# Autodesk Inventor assembly: GANTRY
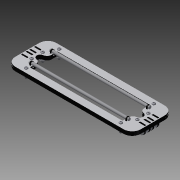
[picture p0: Inventor's stored thumbnail of the model, 180x180]
Saved by Autodesk Inventor 2013 (Build 170138000, 138)
## iProperties
Created: 2014-06-21
Part Number: GANTRY
Document SubType Name: Assembly
Designer: employee
Author: employee
## Documents named in this file (11)
- C:\Users\employee\Desktop\CoreXZ 2\GANTRY.iam
- C:\Users\employee\Desktop\CoreXZ 2\GANTRY BACK.ipt
- C:\Users\employee\Desktop\CoreXZ 2\GANTRY FRONT.ipt
- C:\Users\employee\Desktop\CoreXZ 2\M8X290 ROD.ipt
- C:\Users\employee\Desktop\CoreXZ 2\LM8UU.ipt
- C:\Users\employee\Desktop\CoreXZ 2\625vv.ipt
- C:\Users\employee\Desktop\CoreXZ 2\M5 WASHER.ipt
- C:\Users\employee\Desktop\CoreXZ 2\M5 NUT.ipt
- C:\Users\employee\Desktop\CoreXZ 2\M5X25.ipt
- C:\Users\employee\Desktop\CoreXZ 2\ZIP TIE GANTRY ROD.ipt
- C:\Users\employee\Desktop\CoreXZ 2\ZIP TIE GANTRY BEARING.ipt
## Components (52 placed, 10 different names)
1. GANTRY BACK:1 — Insert:1, Insert:2, Mate:4, Mate:5, Tangent:5, Tangent:6, Tangent:7, Tangent:8, Angle:5, Angle:6, Angle:7, Angle:8, Angle:9, Angle:10, Angle:11, Angle:12, Insert:65, Insert:66, Insert:67, Insert:68, Insert:69, Insert:70, Insert:71, Insert:72
2. GANTRY FRONT:1 — Insert:1, Insert:2, Mate:2, Tangent:1, Tangent:2, Mate:3, Tangent:3, Tangent:4, Angle:1, Angle:2, Angle:3, Angle:4, Insert:73, Insert:74, Insert:75, Insert:76, Insert:77, Insert:78, Insert:79, Insert:80
3. M8X290 ROD:2 — Mate:2, Tangent:1, Tangent:2, Insert:38, Insert:40
4. M8X290 ROD:3 — Mate:3, Tangent:3, Tangent:4, Insert:37, Insert:39
5. LM8UU:1 — Insert:35, Mate:4, Tangent:7, Tangent:8, Insert:47, Insert:48
6. LM8UU:2 — Insert:35, Insert:45, Insert:46
7. LM8UU:3 — Insert:36, Mate:5, Tangent:5, Tangent:6, Insert:43, Insert:44
8. LM8UU:4 — Insert:36, Insert:41, Insert:42
9. ZIP TIE GANTRY ROD:1 — Insert:37, Angle:3
10. ZIP TIE GANTRY ROD:2 — Insert:40, Angle:2
11. ZIP TIE GANTRY ROD:3 — Insert:39, Angle:1
12. ZIP TIE GANTRY ROD:4 — Insert:38, Angle:4
13. ZIP TIE GANTRY BEARING:1 — Insert:41, Angle:5
14. ZIP TIE GANTRY BEARING:2 — Insert:42, Angle:6
15. ZIP TIE GANTRY BEARING:3 — Insert:43, Angle:8
16. ZIP TIE GANTRY BEARING:4 — Insert:44, Angle:7
17. ZIP TIE GANTRY BEARING:5 — Insert:45, Angle:12
18. ZIP TIE GANTRY BEARING:6 — Insert:46, Angle:11
19. ZIP TIE GANTRY BEARING:7 — Insert:47, Angle:9
20. ZIP TIE GANTRY BEARING:8 — Insert:48, Angle:10
21. 625vv:1 — Insert:49, Insert:57
22. M5 NUT:1 — Insert:57
23. M5 WASHER:1 — Insert:49, Insert:65
24. 625vv:2 — Insert:50, Insert:58
25. M5 NUT:2 — Insert:58
26. M5 WASHER:2 — Insert:50, Insert:66
27. 625vv:3 — Insert:51, Insert:59
28. M5 NUT:3 — Insert:59
29. M5 WASHER:3 — Insert:51, Insert:67
30. 625vv:4 — Insert:52, Insert:60
31. M5 NUT:4 — Insert:60
32. M5 WASHER:4 — Insert:52, Insert:68
33. 625vv:5 — Insert:53, Insert:61
34. M5 NUT:5 — Insert:61
35. M5 WASHER:5 — Insert:53, Insert:69
36. 625vv:6 — Insert:54, Insert:62
37. M5 NUT:6 — Insert:62
38. M5 WASHER:6 — Insert:54, Insert:70
39. 625vv:7 — Insert:55, Insert:63
40. M5 NUT:7 — Insert:63
41. M5 WASHER:7 — Insert:55, Insert:71
42. 625vv:8 — Insert:56, Insert:64
43. M5 NUT:8 — Insert:64
44. M5 WASHER:8 — Insert:56, Insert:72
45. M5X25:1 — Insert:73
46. M5X25:2 — Insert:74
47. M5X25:3 — Insert:75
48. M5X25:4 — Insert:76
49. M5X25:5 — Insert:77
50. M5X25:6 — Insert:78
51. M5X25:7 — Insert:79
52. M5X25:8 — Insert:80
## Relationships (72: Insert 48, Angle 12, Tangent 8, Mate 4)
- Insert:1: GANTRY BACK:1 ↔ GANTRY FRONT:1
- Insert:2: GANTRY BACK:1 ↔ GANTRY FRONT:1
- Mate:2: GANTRY FRONT:1 ↔ M8X290 ROD:2
- Tangent:1: GANTRY FRONT:1 ↔ M8X290 ROD:2
- Tangent:2: GANTRY FRONT:1 ↔ M8X290 ROD:2
- Mate:3: GANTRY FRONT:1 ↔ M8X290 ROD:3
- Tangent:3: GANTRY FRONT:1 ↔ M8X290 ROD:3
- Tangent:4: GANTRY FRONT:1 ↔ M8X290 ROD:3
- Insert:35: LM8UU:1 ↔ LM8UU:2
- Insert:36: LM8UU:3 ↔ LM8UU:4
- Mate:4: GANTRY BACK:1 ↔ LM8UU:1
- Mate:5: GANTRY BACK:1 ↔ LM8UU:3
- Tangent:5: GANTRY BACK:1 ↔ LM8UU:3
- Tangent:6: GANTRY BACK:1 ↔ LM8UU:3
- Tangent:7: GANTRY BACK:1 ↔ LM8UU:1
- Tangent:8: GANTRY BACK:1 ↔ LM8UU:1
- Insert:37 (3.25 mm): M8X290 ROD:3 ↔ ZIP TIE GANTRY ROD:1
- Insert:38 (3.25 mm): M8X290 ROD:2 ↔ ZIP TIE GANTRY ROD:4
- Insert:39 (3.25 mm): M8X290 ROD:3 ↔ ZIP TIE GANTRY ROD:3
- Insert:40 (3.25 mm): M8X290 ROD:2 ↔ ZIP TIE GANTRY ROD:2
- Angle:1 (0 deg): GANTRY FRONT:1 ↔ ZIP TIE GANTRY ROD:3
- Angle:2 (0 deg): GANTRY FRONT:1 ↔ ZIP TIE GANTRY ROD:2
- Angle:3 (0 deg): GANTRY FRONT:1 ↔ ZIP TIE GANTRY ROD:1
- Angle:4 (0 deg): GANTRY FRONT:1 ↔ ZIP TIE GANTRY ROD:4
- Insert:41 (3.25 mm): LM8UU:4 ↔ ZIP TIE GANTRY BEARING:1
- Insert:42 (17.25 mm): LM8UU:4 ↔ ZIP TIE GANTRY BEARING:2
- Insert:43 (3.25 mm): LM8UU:3 ↔ ZIP TIE GANTRY BEARING:3
- Insert:44 (17.25 mm): LM8UU:3 ↔ ZIP TIE GANTRY BEARING:4
- Angle:5 (0 deg): GANTRY BACK:1 ↔ ZIP TIE GANTRY BEARING:1
- Angle:6 (0 deg): GANTRY BACK:1 ↔ ZIP TIE GANTRY BEARING:2
- Angle:7 (0 deg): GANTRY BACK:1 ↔ ZIP TIE GANTRY BEARING:4
- Angle:8 (0 deg): GANTRY BACK:1 ↔ ZIP TIE GANTRY BEARING:3
- Insert:45 (3.25 mm): LM8UU:2 ↔ ZIP TIE GANTRY BEARING:5
- Insert:46 (17.25 mm): LM8UU:2 ↔ ZIP TIE GANTRY BEARING:6
- Insert:47 (3.25 mm): LM8UU:1 ↔ ZIP TIE GANTRY BEARING:7
- Insert:48 (17.25 mm): LM8UU:1 ↔ ZIP TIE GANTRY BEARING:8
- Angle:9 (0 deg): GANTRY BACK:1 ↔ ZIP TIE GANTRY BEARING:7
- Angle:10 (0 deg): GANTRY BACK:1 ↔ ZIP TIE GANTRY BEARING:8
- Angle:11 (0 deg): GANTRY BACK:1 ↔ ZIP TIE GANTRY BEARING:6
- Angle:12 (0 deg): GANTRY BACK:1 ↔ ZIP TIE GANTRY BEARING:5
- Insert:49: 625vv:1 ↔ M5 WASHER:1
- Insert:50: 625vv:2 ↔ M5 WASHER:2
- Insert:51: 625vv:3 ↔ M5 WASHER:3
- Insert:52: 625vv:4 ↔ M5 WASHER:4
- Insert:53: 625vv:5 ↔ M5 WASHER:5
- Insert:54: 625vv:6 ↔ M5 WASHER:6
- Insert:55: 625vv:7 ↔ M5 WASHER:7
- Insert:56: 625vv:8 ↔ M5 WASHER:8
- Insert:57: 625vv:1 ↔ M5 NUT:1
- Insert:58: 625vv:2 ↔ M5 NUT:2
- Insert:59: 625vv:3 ↔ M5 NUT:3
- Insert:60: 625vv:4 ↔ M5 NUT:4
- Insert:61: 625vv:5 ↔ M5 NUT:5
- Insert:62: 625vv:6 ↔ M5 NUT:6
- Insert:63: 625vv:7 ↔ M5 NUT:7
- Insert:64: 625vv:8 ↔ M5 NUT:8
- Insert:65: GANTRY BACK:1 ↔ M5 WASHER:1
- Insert:66: GANTRY BACK:1 ↔ M5 WASHER:2
- Insert:67: GANTRY BACK:1 ↔ M5 WASHER:3
- Insert:68: GANTRY BACK:1 ↔ M5 WASHER:4
- Insert:69: GANTRY BACK:1 ↔ M5 WASHER:5
- Insert:70: GANTRY BACK:1 ↔ M5 WASHER:6
- Insert:71: GANTRY BACK:1 ↔ M5 WASHER:7
- Insert:72: GANTRY BACK:1 ↔ M5 WASHER:8
- Insert:73: GANTRY FRONT:1 ↔ M5X25:1
- Insert:74: GANTRY FRONT:1 ↔ M5X25:2
- Insert:75: GANTRY FRONT:1 ↔ M5X25:3
- Insert:76: GANTRY FRONT:1 ↔ M5X25:4
- Insert:77: GANTRY FRONT:1 ↔ M5X25:5
- Insert:78: GANTRY FRONT:1 ↔ M5X25:6
- Insert:79: GANTRY FRONT:1 ↔ M5X25:7
- Insert:80: GANTRY FRONT:1 ↔ M5X25:8
